# Autodesk Inventor assembly: Intake Pivot Encoder Mount
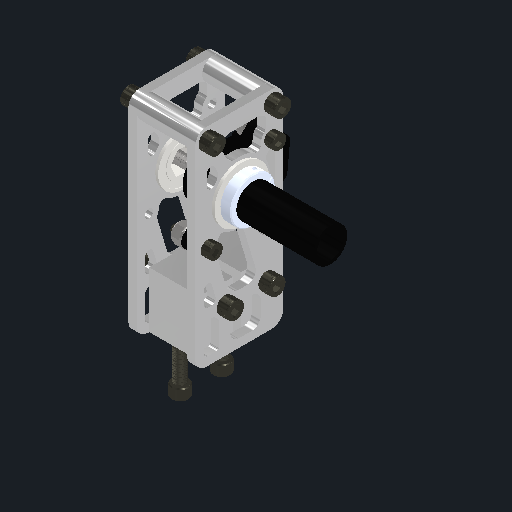
[picture p0: Inventor's stored thumbnail of the model, 512x512]
Saved by Autodesk Inventor 2024.2 (Build 282272000, 272)
## iProperties
Created: 2024-08-03
Part Number: Intake Pivot Encoder Mount
Document SubType Name: Assembly
Designer: Kenji
Mass: 361.107 g
Surface Area: 776.672 cm^2
Volume: 107.275 cm^3
Density: 3.36617 g/cm^3
Author: Kenji
## Documents named in this file (15)
- C:\Users\bobsb\OneDrive\Documents\GitHub\1622-2024-Summer-CAD-A-Thon\Intake\Intake Pivot Encoder Mount.iam
- C:\Users\bobsb\OneDrive\Documents\GitHub\1622-2024-Summer-CAD-A-Thon\Intake\Intake Pivot Spacer 3.ipt
- C:\Users\bobsb\OneDrive\Documents\GitHub\1622-2024-Summer-CAD-A-Thon\Intake\Intake Pivot Billet.ipt
- C:\Users\bobsb\OneDrive\Documents\GitHub\1622-2024-Summer-CAD-A-Thon\COTS Library\Fasteners\Bolts\Socket-Head\0.25-20\COTS_91251A539_Black-Oxide Alloy Steel Socket Head Screw (1).ipt
- C:\Users\bobsb\OneDrive\Documents\GitHub\1622-2024-Summer-CAD-A-Thon\COTS Library\Motion\Bearings\COTS_WCP-0783_1.125ODHexBearing.ipt
- C:\Users\bobsb\OneDrive\Documents\GitHub\1622-2024-Summer-CAD-A-Thon\COTS Library\Fasteners\Bolts\Button-Head\0.25-20\COTS_0.25-20_ButtonHead_0.5inlong_StainlessSteel_92949A537.ipt
- C:\Users\bobsb\OneDrive\Documents\GitHub\1622-2024-Summer-CAD-A-Thon\COTS Library\Fasteners\Washers\COTS_90107A029_316 Stainless Steel Washer.ipt
- C:\Users\bobsb\OneDrive\Documents\GitHub\1622-2024-Summer-CAD-A-Thon\COTS Library\Fasteners\Nuts\COTS_90631A411_10-32_Nylock_Nut.ipt
- C:\Users\bobsb\OneDrive\Documents\GitHub\1622-2024-Summer-CAD-A-Thon\COTS Library\Fasteners\Washers\COTS_91860A047_Size10Washer.ipt
- C:\Users\bobsb\OneDrive\Documents\GitHub\1622-2024-Summer-CAD-A-Thon\COTS Library\Fasteners\Bolts\Socket-Head\10-32\COTS_91251A345_Black-Oxide Alloy Steel Socket Head Screw.ipt
- C:\Users\bobsb\OneDrive\Documents\GitHub\1622-2024-Summer-CAD-A-Thon\COTS Library\Fasteners\Shaft Collars\COTS_WCP-0799_0.5inchHexShaftCollar.ipt
- C:\Users\bobsb\OneDrive\Documents\GitHub\1622-2024-Summer-CAD-A-Thon\Intake\Intake Pivot Spacer 4.ipt
- C:\Users\bobsb\OneDrive\Documents\GitHub\1622-2024-Summer-CAD-A-Thon\COTS Library\Fasteners\Bolts\Socket-Head\0.25-20\COTS_90044A123_Black-Oxide Alloy Steel Socket Head Screw.ipt
- C:\Users\bobsb\OneDrive\Documents\GitHub\1622-2024-Summer-CAD-A-Thon\COTS Library\Electrical Components\REV\COTS_REV-11-1271_ThroughBoreEncoder.iam
- C:\Users\bobsb\OneDrive\Documents\GitHub\1622-2024-Summer-CAD-A-Thon\Intake\INTK_008_EncoderBracket.ipt
## Components (29 placed, 14 different names)
1. Intake Pivot Spacer 3:1 — Mate:86, Mate:87
2. Intake Pivot Spacer 3:2 — Mate:83, Mate:84, Mate:85
3. Intake Pivot Billet:1 — Mate:61, Mate:64, Mate:96, Mate:97, Flush:1
4. Intake Pivot Billet:2 — Mate:62, Mate:63, Mate:102, Mate:103, Flush:2
5. COTS_91251A539_Black-Oxide Alloy Steel Socket Head Screw (1):1 — Mate:93, Mate:95
6. COTS_91251A539_Black-Oxide Alloy Steel Socket Head Screw (1):2 — Mate:88, Mate:90
7. COTS_91251A539_Black-Oxide Alloy Steel Socket Head Screw (1):3 — Mate:92, Mate:94
8. COTS_91251A539_Black-Oxide Alloy Steel Socket Head Screw (1):4 — Mate:89, Mate:91
9. COTS_91251A539_Black-Oxide Alloy Steel Socket Head Screw (1):5 — Mate:105, Mate:106
10. COTS_91251A539_Black-Oxide Alloy Steel Socket Head Screw (1):6 — Mate:104, Mate:107
11. COTS_91251A539_Black-Oxide Alloy Steel Socket Head Screw (1):7 — Mate:99, Mate:100
12. COTS_91251A539_Black-Oxide Alloy Steel Socket Head Screw (1):8 — Mate:98, Mate:101
13. COTS_WCP-0783_1.125ODHexBearing:1 — Mate:30, Mate:31, Mate:81, Mate:82
14. COTS_0.25-20_ButtonHead_0.5inlong_StainlessSteel_92949A537:1 — Mate:32, Mate:33
15. COTS_90107A029_316 Stainless Steel Washer:1 — Mate:30, Mate:31, Mate:32, Mate:33
16. COTS_90631A411_10-32_Nylock_Nut:1 — Mate:49, Mate:50
17. COTS_90631A411_10-32_Nylock_Nut:2 — Mate:47, Mate:48
18. COTS_91860A047_Size10Washer:1 — Mate:49, Mate:50, Mate:69, Mate:80
19. COTS_91860A047_Size10Washer:2 — Mate:47, Mate:48, Mate:68, Mate:79
20. COTS_91251A345_Black-Oxide Alloy Steel Socket Head Screw:1 — Mate:77, Mate:78, Mate:79
21. COTS_91251A345_Black-Oxide Alloy Steel Socket Head Screw:2 — Mate:66, Mate:76, Mate:80
22. COTS_WCP-0783_1.125ODHexBearing:2 — Mate:57, Mate:58, Mate:65, Mate:72, Mate:73
23. COTS_WCP-0799_0.5inchHexShaftCollar:1 — Mate:57, Mate:58, Mate:59, Mate:60
24. Intake Pivot Spacer 4:1 — Mate:59, Mate:60
25. COTS_90044A123_Black-Oxide Alloy Steel Socket Head Screw:1 — Mate:61, Mate:64
26. COTS_90044A123_Black-Oxide Alloy Steel Socket Head Screw:2 — Mate:62, Mate:63
27. COTS_REV-11-1271_ThroughBoreEncoder:1 [sub-assembly] — Mate:65, Mate:66, Mate:68, Mate:69, Mate:74, Mate:75
28. INTK_008_EncoderBracket:1 — Mate:70, Mate:71, Mate:81, Mate:82, Mate:84, Mate:87, Mate:89, Mate:91, Mate:93, Mate:95, Mate:99, Mate:100, Mate:105, Mate:106
29. INTK_008_EncoderBracket:2 — Mate:70, Mate:71, Mate:72, Mate:73, Mate:74, Mate:75, Mate:76, Mate:77, Mate:78, Mate:83, Mate:85, Mate:86, Mate:88, Mate:90, Mate:92, Mate:94, Mate:96, Mate:97, Flush:1, Mate:98, Mate:101, Mate:102, Mate:103, Flush:2, Mate:104, Mate:107
## Relationships (60: Mate 58, Flush 2)
- Mate:30: COTS_WCP-0783_1.125ODHexBearing:1 ↔ COTS_90107A029_316 Stainless Steel Washer:1
- Mate:31: COTS_WCP-0783_1.125ODHexBearing:1 ↔ COTS_90107A029_316 Stainless Steel Washer:1
- Mate:32: COTS_0.25-20_ButtonHead_0.5inlong_StainlessSteel_92949A537:1 ↔ COTS_90107A029_316 Stainless Steel Washer:1
- Mate:33: COTS_0.25-20_ButtonHead_0.5inlong_StainlessSteel_92949A537:1 ↔ COTS_90107A029_316 Stainless Steel Washer:1
- Mate:47: COTS_90631A411_10-32_Nylock_Nut:2 ↔ COTS_91860A047_Size10Washer:2
- Mate:48: COTS_90631A411_10-32_Nylock_Nut:2 ↔ COTS_91860A047_Size10Washer:2
- Mate:49: COTS_90631A411_10-32_Nylock_Nut:1 ↔ COTS_91860A047_Size10Washer:1
- Mate:50: COTS_90631A411_10-32_Nylock_Nut:1 ↔ COTS_91860A047_Size10Washer:1
- Mate:57: COTS_WCP-0783_1.125ODHexBearing:2 ↔ COTS_WCP-0799_0.5inchHexShaftCollar:1
- Mate:58: COTS_WCP-0783_1.125ODHexBearing:2 ↔ COTS_WCP-0799_0.5inchHexShaftCollar:1
- Mate:59: COTS_WCP-0799_0.5inchHexShaftCollar:1 ↔ Intake Pivot Spacer 4:1
- Mate:60: COTS_WCP-0799_0.5inchHexShaftCollar:1 ↔ Intake Pivot Spacer 4:1
- Mate:61: Intake Pivot Billet:1 ↔ COTS_90044A123_Black-Oxide Alloy Steel Socket Head Screw:1
- Mate:62: Intake Pivot Billet:2 ↔ COTS_90044A123_Black-Oxide Alloy Steel Socket Head Screw:2
- Mate:63 (25.4 mm): Intake Pivot Billet:2 ↔ COTS_90044A123_Black-Oxide Alloy Steel Socket Head Screw:2
- Mate:64 (25.4 mm): Intake Pivot Billet:1 ↔ COTS_90044A123_Black-Oxide Alloy Steel Socket Head Screw:1
- Mate:65: COTS_WCP-0783_1.125ODHexBearing:2 ↔ COTS_REV-11-1271_ThroughBoreEncoder:1
- Mate:66: COTS_91251A345_Black-Oxide Alloy Steel Socket Head Screw:2 ↔ COTS_REV-11-1271_ThroughBoreEncoder:1
- Mate:68: COTS_91860A047_Size10Washer:2 ↔ COTS_REV-11-1271_ThroughBoreEncoder:1
- Mate:69: COTS_91860A047_Size10Washer:1 ↔ COTS_REV-11-1271_ThroughBoreEncoder:1
- Mate:70: INTK_008_EncoderBracket:1 ↔ INTK_008_EncoderBracket:2
- Mate:71: INTK_008_EncoderBracket:1 ↔ INTK_008_EncoderBracket:2
- Mate:72: COTS_WCP-0783_1.125ODHexBearing:2 ↔ INTK_008_EncoderBracket:2
- Mate:73: COTS_WCP-0783_1.125ODHexBearing:2 ↔ INTK_008_EncoderBracket:2
- Mate:74: COTS_REV-11-1271_ThroughBoreEncoder:1 ↔ INTK_008_EncoderBracket:2
- Mate:75: COTS_REV-11-1271_ThroughBoreEncoder:1 ↔ INTK_008_EncoderBracket:2
- Mate:76: COTS_91251A345_Black-Oxide Alloy Steel Socket Head Screw:2 ↔ INTK_008_EncoderBracket:2
- Mate:77: COTS_91251A345_Black-Oxide Alloy Steel Socket Head Screw:1 ↔ INTK_008_EncoderBracket:2
- Mate:78: COTS_91251A345_Black-Oxide Alloy Steel Socket Head Screw:1 ↔ INTK_008_EncoderBracket:2
- Mate:79: COTS_91860A047_Size10Washer:2 ↔ COTS_91251A345_Black-Oxide Alloy Steel Socket Head Screw:1
- Mate:80: COTS_91860A047_Size10Washer:1 ↔ COTS_91251A345_Black-Oxide Alloy Steel Socket Head Screw:2
- Mate:81: COTS_WCP-0783_1.125ODHexBearing:1 ↔ INTK_008_EncoderBracket:1
- Mate:82: COTS_WCP-0783_1.125ODHexBearing:1 ↔ INTK_008_EncoderBracket:1
- Mate:83: Intake Pivot Spacer 3:2 ↔ INTK_008_EncoderBracket:2
- Mate:84: Intake Pivot Spacer 3:2 ↔ INTK_008_EncoderBracket:1
- Mate:85: Intake Pivot Spacer 3:2 ↔ INTK_008_EncoderBracket:2
- Mate:86: Intake Pivot Spacer 3:1 ↔ INTK_008_EncoderBracket:2
- Mate:87: Intake Pivot Spacer 3:1 ↔ INTK_008_EncoderBracket:1
- Mate:88: COTS_91251A539_Black-Oxide Alloy Steel Socket Head Screw (1):2 ↔ INTK_008_EncoderBracket:2
- Mate:89: COTS_91251A539_Black-Oxide Alloy Steel Socket Head Screw (1):4 ↔ INTK_008_EncoderBracket:1
- Mate:90: COTS_91251A539_Black-Oxide Alloy Steel Socket Head Screw (1):2 ↔ INTK_008_EncoderBracket:2
- Mate:91: COTS_91251A539_Black-Oxide Alloy Steel Socket Head Screw (1):4 ↔ INTK_008_EncoderBracket:1
- Mate:92: COTS_91251A539_Black-Oxide Alloy Steel Socket Head Screw (1):3 ↔ INTK_008_EncoderBracket:2
- Mate:93: COTS_91251A539_Black-Oxide Alloy Steel Socket Head Screw (1):1 ↔ INTK_008_EncoderBracket:1
- Mate:94: COTS_91251A539_Black-Oxide Alloy Steel Socket Head Screw (1):3 ↔ INTK_008_EncoderBracket:2
- Mate:95: COTS_91251A539_Black-Oxide Alloy Steel Socket Head Screw (1):1 ↔ INTK_008_EncoderBracket:1
- Mate:96: Intake Pivot Billet:1 ↔ INTK_008_EncoderBracket:2
- Mate:97: Intake Pivot Billet:1 ↔ INTK_008_EncoderBracket:2
- Flush:1: Intake Pivot Billet:1 ↔ INTK_008_EncoderBracket:2
- Mate:98: COTS_91251A539_Black-Oxide Alloy Steel Socket Head Screw (1):8 ↔ INTK_008_EncoderBracket:2
- Mate:99: COTS_91251A539_Black-Oxide Alloy Steel Socket Head Screw (1):7 ↔ INTK_008_EncoderBracket:1
- Mate:100: COTS_91251A539_Black-Oxide Alloy Steel Socket Head Screw (1):7 ↔ INTK_008_EncoderBracket:1
- Mate:101: COTS_91251A539_Black-Oxide Alloy Steel Socket Head Screw (1):8 ↔ INTK_008_EncoderBracket:2
- Mate:102: Intake Pivot Billet:2 ↔ INTK_008_EncoderBracket:2
- Mate:103: Intake Pivot Billet:2 ↔ INTK_008_EncoderBracket:2
- Flush:2: Intake Pivot Billet:2 ↔ INTK_008_EncoderBracket:2
- Mate:104: COTS_91251A539_Black-Oxide Alloy Steel Socket Head Screw (1):6 ↔ INTK_008_EncoderBracket:2
- Mate:105: COTS_91251A539_Black-Oxide Alloy Steel Socket Head Screw (1):5 ↔ INTK_008_EncoderBracket:1
- Mate:106: COTS_91251A539_Black-Oxide Alloy Steel Socket Head Screw (1):5 ↔ INTK_008_EncoderBracket:1
- Mate:107: COTS_91251A539_Black-Oxide Alloy Steel Socket Head Screw (1):6 ↔ INTK_008_EncoderBracket:2
